# Autodesk Inventor assembly: KTN_MultiPass
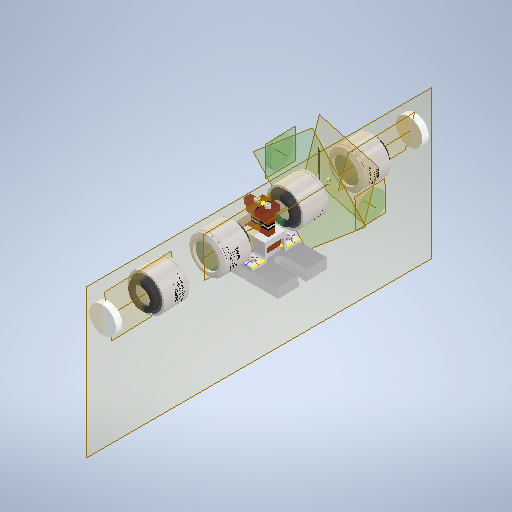
[picture p0: Inventor's stored thumbnail of the model, 512x512]
Saved by Autodesk Inventor 2025 (Build 290162010, 162A)
## iProperties
Created: 2024-04-24
Part Number: KTN_MultiPass
Document SubType Name: Assembly
Designer: kerlin
Author: kerlin
## Documents named in this file (8)
- C:\Users\User\Desktop\Hari_Laptop_Contents\KerlinLab\KTN\Multipass\MechanicalDrawing\KTN_MultiPass.iam
- C:\Users\User\Desktop\Hari_Laptop_Contents\KerlinLab\KTN\Multipass\MechanicalDrawing\LSM03-BB-Solidworks.ipt
- C:\Users\User\Desktop\Hari_Laptop_Contents\KerlinLab\KTN\Multipass\MechanicalDrawing\BB1-E02-Solidworks.ipt
- C:\Users\User\Desktop\Hari_Laptop_Contents\KerlinLab\KTN\Multipass\MechanicalDrawing\MRA03-P01-Solidworks.ipt
- C:\Users\User\Desktop\Hari_Laptop_Contents\KerlinLab\KTN\Multipass\MechanicalDrawing\pckngo_D1\EOD_D1_v2.0.iam
- C:\Users\User\Desktop\Hari_Laptop_Contents\KerlinLab\KTN\Multipass\MechanicalDrawing\ExitMirror.ipt
- C:\Users\User\Desktop\Hari_Laptop_Contents\KerlinLab\KTN\Multipass\MechanicalDrawing\CylConcaveLens.ipt
- C:\Users\User\Desktop\Hari_Laptop_Contents\KerlinLab\KTN\Multipass\MechanicalDrawing\Lens.ipt
## Components (12 placed, 7 different names)
1. LSM03-BB-Solidworks:1 — Mate:3, Mate:4, Mate:5, Mate:6, Angle:2, Mate:13, Flush:6, Mate:14
2. LSM03-BB-Solidworks:2 — Mate:3, Mate:6, Mate:9, Mate:10
3. LSM03-BB-Solidworks:3 — Mate:1, Mate:7, Mate:8, Mate:11, Flush:4
4. LSM03-BB-Solidworks:4 — Mate:1, Mate:4, Mate:5, Mate:7, Flush:5
5. BB1-E02-Solidworks:1 — Mate:8, Mate:11, Mate:12
6. BB1-E02-Solidworks:2 — Mate:9, Mate:10
7. MRA03-P01-Solidworks:1 — Mate:12, Angle:1, Mate:14, Mate:15, Mate:16
8. EOD_D1_v2.0:1 [sub-assembly] — Flush:2
9. ExitMirror:1 — Angle:1
10. CylConcaveLens:1
11. Lens:1 — Mate:15
12. Lens:2 — Mate:16
## Relationships (21: Mate 15, Flush 4, Angle 2)
- Mate:1: LSM03-BB-Solidworks:3 ↔ LSM03-BB-Solidworks:4
- Mate:3: LSM03-BB-Solidworks:1 ↔ LSM03-BB-Solidworks:2
- Mate:4: LSM03-BB-Solidworks:1 ↔ LSM03-BB-Solidworks:4
- Mate:5 (40 mm): LSM03-BB-Solidworks:1 ↔ LSM03-BB-Solidworks:4
- Mate:6 (30 mm): LSM03-BB-Solidworks:1 ↔ LSM03-BB-Solidworks:2
- Mate:7 (30 mm): LSM03-BB-Solidworks:3 ↔ LSM03-BB-Solidworks:4
- Mate:8: LSM03-BB-Solidworks:3 ↔ BB1-E02-Solidworks:1
- Mate:9: LSM03-BB-Solidworks:2 ↔ BB1-E02-Solidworks:2
- Mate:10 (30 mm): LSM03-BB-Solidworks:2 ↔ BB1-E02-Solidworks:2
- Mate:11 (30 mm): LSM03-BB-Solidworks:3 ↔ BB1-E02-Solidworks:1
- Mate:12 (-82 mm): BB1-E02-Solidworks:1 ↔ MRA03-P01-Solidworks:1
- Angle:1 (0 deg): MRA03-P01-Solidworks:1 ↔ ExitMirror:1
- Angle:2 (0 deg): LSM03-BB-Solidworks:1
- Flush:2 (28 mm): EOD_D1_v2.0:1
- Mate:13: LSM03-BB-Solidworks:1
- Flush:4: LSM03-BB-Solidworks:3
- Flush:5: LSM03-BB-Solidworks:4
- Flush:6: LSM03-BB-Solidworks:1
- Mate:14: LSM03-BB-Solidworks:1 ↔ MRA03-P01-Solidworks:1
- Mate:15: MRA03-P01-Solidworks:1 ↔ Lens:1
- Mate:16: MRA03-P01-Solidworks:1 ↔ Lens:2
